# Autodesk Inventor assembly: Montiert
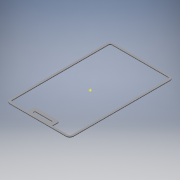
[picture p0: Inventor's stored thumbnail of the model, 180x180]
Saved by Autodesk Inventor 2018 (Build 220112000, 112)
## iProperties
Created: 2017-11-12
Part Number: Montiert
Material: Generisch
Document SubType Name: Assembly
## Documents named in this file (2)
- C:\git\RoKu-ProjectX01\Konstruktion\Montiert.iam
- C:\git\RoKu-ProjectX01\Konstruktion\Rost_Basis.ipt
## Components (1 placed, 1 different names)
1. Rost_Basis:1 — Fluchtend:1, Fluchtend:2, Fluchtend:3
## Relationships (3: Flush 3)
- Fluchtend:1 [Flush]: Rost_Basis:1
- Fluchtend:2 [Flush]: Rost_Basis:1
- Fluchtend:3 [Flush]: Rost_Basis:1
